# Autodesk Inventor assembly: main
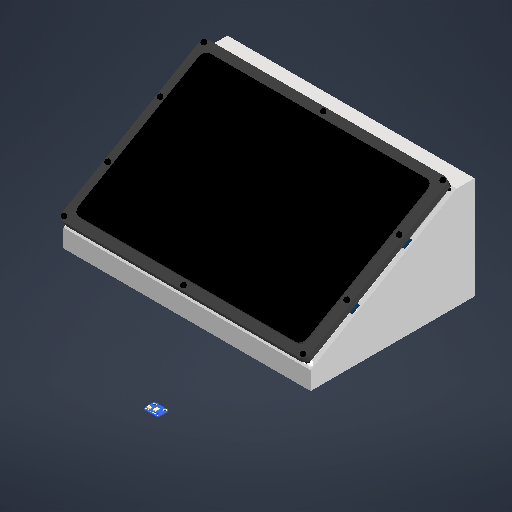
[picture p0: Inventor's stored thumbnail of the model, 512x512]
Saved by Autodesk Inventor 2026.2 (Build 302298000, 298)
## iProperties
Created: 2025-12-22
Part Number: main
Document SubType Name: Assembly
Designer: test
wood_thickness: 10.000 mm
Author: test
## Documents named in this file (5)
- C:\Users\test\Projects\simple-concert-monitor\simple-concert-monitor_Mechanical\main.iam
- C:\Users\test\Projects\simple-concert-monitor\simple-concert-monitor_Mechanical\screen\screen.iam
- C:\Users\test\Projects\simple-concert-monitor\simple-concert-monitor_Mechanical\external\raspberry-pi-4-model-b-1.snapshot.3\Raspberry Pi 4 Model B\Raspberry Pi 4 Model B\Raspberry Pi 4 Model B.iam
- C:\Users\test\Projects\simple-concert-monitor\simple-concert-monitor_Mechanical\case1.ipt
- C:\Users\test\Projects\simple-concert-monitor\simple-concert-monitor_Mechanical\external\adafruit-i2s-pi-mic-breakout-sph0645-1.snapshot.1\Pi Mic breakout SPH0645\Pi Mic breakout SPH0645\Pi Mic breakout SPH0645.ipt
## Components (4 placed, 4 different names)
1. screen:1 [sub-assembly] — Mate:2, Angle:1
2. Raspberry Pi 4 Model B:1 [sub-assembly]
3. case1:1 — Mate:1, Mate:2, Angle:1
4. Pi Mic breakout SPH0645:1
## Relationships (3: Mate 2, Angle 1)
- Mate:1: case1:1
- Mate:2: screen:1 ↔ case1:1
- Angle:1 (0 deg): screen:1 ↔ case1:1
